# Autodesk Inventor assembly: Backplane
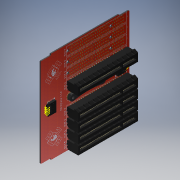
[picture p0: Inventor's stored thumbnail of the model, 180x180]
Saved by Autodesk Inventor 2018 (Build 220112000, 112)
## iProperties
Created: 2018-10-18
Part Number: Backplane
Document SubType Name: Assembly
Designer: Bradley
Author: Bradley
## Documents named in this file (8)
- C:\Users\Bradley\Documents\GitHub\CougsInSpace\CougSat1-Hardware\CougSat1-Backplane\CADModel\Native\Backplane.iam
- C:\Users\Bradley\Documents\GitHub\CougsInSpace\CougSat1-Hardware\CougSat1-Backplane\CADModel\Native\Backplane_PCB.ipt
- C:\Users\Bradley\Documents\GitHub\CougsInSpace\Resources\ComponentModels\Connectors\PicoLock-J-4.ipt
- C:\Users\Bradley\Documents\GitHub\CougsInSpace\Resources\ComponentModels\Connectors\PicoLock-P-4.ipt
- C:\Users\Bradley\Documents\GitHub\CougsInSpace\Resources\ComponentModels\Electronics\Capacitor_1608-0.8mm.ipt
- C:\Users\Bradley\Documents\GitHub\CougsInSpace\Resources\ComponentModels\Electronics\Resistor_1608-0.5mm.ipt
- C:\Users\Bradley\Documents\GitHub\CougsInSpace\CougSat1-Hardware\CougSat1-Backplane\CADModel\Native\Backplane_CenterNut.ipt
- C:\Users\Bradley\Documents\GitHub\CougsInSpace\Resources\ComponentModels\Connectors\PCIe-x8.ipt
## Components (15 placed, 7 different names)
1. Backplane_PCB:1 — Mate:5, Mate:6, Mate:9, Mate:10, Mate:11, Mate:12, Insert:17, Insert:18, Mate:21, Mate:22, Mate:23, Mate:24, Mate:25, Mate:26, Mate:27, Mate:28, Mate:29, Mate:30
2. Backplane_CenterNut:1 — Insert:17, Insert:18
3. PCIe-x8:5 — Mate:25, Mate:26, Angle:5
4. PCIe-x8:4 — Mate:24, Mate:27, Angle:4
5. PCIe-x8:3 — Mate:23, Mate:28, Angle:3
6. PCIe-x8:2 — Mate:22, Mate:29, Angle:2
7. PCIe-x8:1 — Mate:21, Mate:30, Angle:1
8. PicoLock-J-4:1 — Mate:5, Flush:3, Mate:7
9. PicoLock-J-4:2 — Mate:6, Mate:8, Flush:4
10. PicoLock-P-4:1
11. PicoLock-P-4:2
12. Capacitor_1608-0.8mm:1 — Mate:11, Mate:13, Mate:14
13. Capacitor_1608-0.8mm:2 — Mate:12, Mate:17, Mate:18
14. Resistor_1608-0.5mm:1 — Mate:9, Mate:15, Mate:16
15. Resistor_1608-0.5mm:2 — Mate:10, Mate:19, Mate:20
## Relationships (41: Mate 30, Angle 5, Flush 4, Insert 2)
- [Flush]: PicoLock-J-4:1 ↔ PicoLock-P-4:1
- [Mate]: PicoLock-J-4:1 ↔ PicoLock-P-4:1
- [Mate] (0.025 mm): PicoLock-J-4:1 ↔ PicoLock-P-4:1
- [Flush]: PicoLock-J-4:2 ↔ PicoLock-P-4:2
- [Mate]: PicoLock-J-4:2 ↔ PicoLock-P-4:2
- [Mate] (0.025 mm): PicoLock-J-4:2 ↔ PicoLock-P-4:2
- Mate:5: Backplane_PCB:1 ↔ PicoLock-J-4:1
- Mate:6: Backplane_PCB:1 ↔ PicoLock-J-4:2
- Flush:3: PicoLock-J-4:1
- Mate:7 (-29 mm): PicoLock-J-4:1
- Mate:8: PicoLock-J-4:2
- Flush:4 (29 mm): PicoLock-J-4:2
- Mate:9: Backplane_PCB:1 ↔ Resistor_1608-0.5mm:1
- Mate:10: Backplane_PCB:1 ↔ Resistor_1608-0.5mm:2
- Mate:11: Backplane_PCB:1 ↔ Capacitor_1608-0.8mm:1
- Mate:12: Backplane_PCB:1 ↔ Capacitor_1608-0.8mm:2
- Mate:13 (-1.8 mm): Capacitor_1608-0.8mm:1
- Mate:14 (-9.5 mm): Capacitor_1608-0.8mm:1
- Mate:15 (1.8 mm): Resistor_1608-0.5mm:1
- Mate:16 (-9.5 mm): Resistor_1608-0.5mm:1
- Insert:17: Backplane_PCB:1 ↔ Backplane_CenterNut:1
- Insert:18: Backplane_PCB:1 ↔ Backplane_CenterNut:1
- Mate:17 (-1.8 mm): Capacitor_1608-0.8mm:2
- Mate:18 (9.5 mm): Capacitor_1608-0.8mm:2
- Mate:19 (1.8 mm): Resistor_1608-0.5mm:2
- Mate:20 (9.5 mm): Resistor_1608-0.5mm:2
- Mate:21: Backplane_PCB:1 ↔ PCIe-x8:1
- Mate:22: Backplane_PCB:1 ↔ PCIe-x8:2
- Mate:23: Backplane_PCB:1 ↔ PCIe-x8:3
- Mate:24: Backplane_PCB:1 ↔ PCIe-x8:4
- Mate:25: Backplane_PCB:1 ↔ PCIe-x8:5
- Mate:26: Backplane_PCB:1 ↔ PCIe-x8:5
- Mate:27: Backplane_PCB:1 ↔ PCIe-x8:4
- Mate:28: Backplane_PCB:1 ↔ PCIe-x8:3
- Mate:29: Backplane_PCB:1 ↔ PCIe-x8:2
- Mate:30: Backplane_PCB:1 ↔ PCIe-x8:1
- Angle:1 (0 deg): PCIe-x8:1
- Angle:2 (0 deg): PCIe-x8:2
- Angle:3 (0 deg): PCIe-x8:3
- Angle:4 (0 deg): PCIe-x8:4
- Angle:5 (0 deg): PCIe-x8:5
## Named parameters: d3_d9 = 0 mm, d4_d10 = 0 mm, d5_d11 = 0.025 mm
